# Autodesk Inventor assembly: omniwheel_assembly
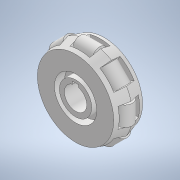
[picture p0: Inventor's stored thumbnail of the model, 180x180]
Saved by Autodesk Inventor 2020.2 (Build 242310000, 310)
## iProperties
Created: 2020-06-12
Part Number: omniwheel_assembly
Document SubType Name: Assembly
Designer: Tarsoly
Author: Tarsoly
## Documents named in this file (3)
- D:\Users\Tarsoly\Dokumentumok\BME\8. Félév\Önlab\3d\omniwheel_assembly.iam
- D:\Users\Tarsoly\Dokumentumok\BME\8. Félév\Önlab\3d\omniwheel.ipt
- D:\Users\Tarsoly\Dokumentumok\BME\8. Félév\Önlab\3d\wheel_little_wheel.ipt
## Components (9 placed, 2 different names)
1. omniwheel:1 — Mate:1, Mate:2, Tangent:1
2. wheel_little_wheel:1 — Mate:3, Mate:7, Mate:8
3. wheel_little_wheel:2
4. wheel_little_wheel:3
5. wheel_little_wheel:4
6. wheel_little_wheel:5
7. wheel_little_wheel:6
8. wheel_little_wheel:7
9. wheel_little_wheel:8
## Component patterns: (8 elements, first: wheel_little_wheel:1)
## Relationships (6: Mate 5, Tangent 1)
- Mate:1: omniwheel:1
- Mate:2: omniwheel:1
- Mate:3: wheel_little_wheel:1
- Mate:7: wheel_little_wheel:1
- Mate:8: wheel_little_wheel:1
- Tangent:1: omniwheel:1
